# Autodesk Inventor assembly: Encrusting Machine
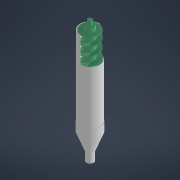
[picture p0: Inventor's stored thumbnail of the model, 180x180]
Saved by Autodesk Inventor 2021 (Build 250183000, 183)
## iProperties
Created: 2022-05-23
Part Number: Encrusting Machine
Document SubType Name: Assembly
Designer: techv
Author: techv
## Documents named in this file (4)
- D:\Projects\P_Baker Bot\Encrusting Machine\Encrusting Machine.iam
- D:\Projects\P_Baker Bot\Encrusting Machine\4.5 to 1.5 inch reducer.ipt
- D:\Projects\P_Baker Bot\Encrusting Machine\4.5 inch diameter pipe.ipt
- D:\Projects\P_Baker Bot\Encrusting Machine\screw_feeder.ipt
## Components (3 placed, 3 different names)
1. 4.5 to 1.5 inch reducer:1 — Mate:1
2. 4.5 inch diameter pipe:1 — Mate:1, Flush:2, Mate:2, Mate:3, Flush:3
3. screw_feeder:1 — Flush:1, Flush:2, Mate:2, Mate:3, Flush:3
## Relationships (6: Flush 3, Mate 3)
- Flush:1 (-135 mm): screw_feeder:1
- Mate:1 (-40 mm): 4.5 to 1.5 inch reducer:1 ↔ 4.5 inch diameter pipe:1
- Flush:2: 4.5 inch diameter pipe:1 ↔ screw_feeder:1
- Mate:2: 4.5 inch diameter pipe:1 ↔ screw_feeder:1
- Mate:3: 4.5 inch diameter pipe:1 ↔ screw_feeder:1
- Flush:3: 4.5 inch diameter pipe:1 ↔ screw_feeder:1
